# Autodesk Inventor assembly: Electrical System
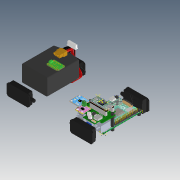
[picture p0: Inventor's stored thumbnail of the model, 180x180]
Saved by Autodesk Inventor 2020 (Build 240168000, 168)
## iProperties
Created: 2020-09-28
Part Number: Electrical System
Document SubType Name: Assembly
Designer: DELL
Mass: 1647.14 g
Surface Area: 7380.95 cm^2
Volume: 1642.04 cm^3
Density: 1.0031 g/cm^3
Author: DELL
## Documents named in this file (5)
- F:\SoftRobot\Model\FlexipodHardware-Zhicheng_09_29_2020\mechanical_model\Electrical System\Electrical System.iam
- F:\SoftRobot\Model\FlexipodHardware-Zhicheng_09_29_2020\mechanical_model\PCB\PCB_board_assembly.iam
- F:\SoftRobot\Model\FlexipodHardware-Zhicheng_09_29_2020\mechanical_model\Electrical System\battery_6s_1550_ovonic.ipt
- F:\SoftRobot\Model\FlexipodHardware-Zhicheng_09_29_2020\mechanical_model\Electrical System\ESC.ipt
- F:\SoftRobot\Model\FlexipodHardware-Zhicheng_09_29_2020\mechanical_model\PCB\Adafruit-LSM6DSOX-LIS3MDL-PCB\Adafruit_LIS3MDL_LSM6DSOX.iam
## Components (7 placed, 4 different names)
1. PCB_board_assembly:1 [sub-assembly]
2. battery_6s_1550_ovonic:1 — Mate:5
3. ESC:1 — Mate:1, Mate:2
4. ESC:2 — Mate:3, Mate:4
5. ESC:4 — Mate:3, Mate:4
6. ESC:5 — Mate:1, Mate:2
7. Adafruit_LIS3MDL_LSM6DSOX:1 [sub-assembly] — Mate:5
## Relationships (5: Mate 5)
- Mate:1: ESC:1 ↔ ESC:5
- Mate:2: ESC:1 ↔ ESC:5
- Mate:3: ESC:2 ↔ ESC:4
- Mate:4: ESC:2 ↔ ESC:4
- Mate:5: battery_6s_1550_ovonic:1 ↔ Adafruit_LIS3MDL_LSM6DSOX:1
